# Autodesk Inventor assembly: FE-00002-11
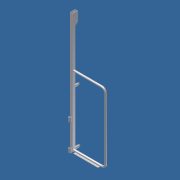
[picture p0: Inventor's stored thumbnail of the model, 180x180]
Saved by Autodesk Inventor 2012 (Build 160160000, 160)
## iProperties
Created: 2008-05-15
Part Number: FE-00002-11
Document SubType Name: Assembly
Designer: narosenberg
Author: narosenberg
## Documents named in this file (8)
- C:\Data Folder\FRC 2012 Field\Components\FE-00002-11.iam
- C:\Data Folder\FRC 2012 Field\Components\FE-00002-01.ipt
- C:\Data Folder\FRC 2012 Field\Components\FE-00002-02.ipt
- C:\Data Folder\FRC 2012 Field\Components\FE-00002-03.ipt
- C:\Data Folder\FRC 2012 Field\Components\FE-00002-05.ipt
- C:\Data Folder\FRC 2012 Field\Components\FE-00002-06.ipt
- C:\Data Folder\FRC 2012 Field\Components\FE-00002-07.ipt
- C:\Data Folder\FRC 2012 Field\Components\FE-00002-09.ipt
## Components (8 placed, 7 different names)
1. FE-00002-06:1 — Mate:1, Tangent:1, Flush:1, Mate:4
2. FE-00002-07:1 — Mate:3, Tangent:1, Flush:1, Flush:2
3. FE-00002-05:1 — Mate:4, Flush:2, Flush:3, Insert:1, Insert:2, Mate:6, Mate:7, Mate:8, Mate:9, Tangent:2, Flush:4
4. FE-00002-01:1 — Insert:1
5. FE-00002-02:1 — Insert:2
6. FE-00002-03:1 — Mate:6, Mate:7
7. FE-00002-09:2 — Mate:12, Tangent:2, Flush:4, Insert:3
8. FE-00002-09:1 — Mate:13, Insert:3
## Relationships (24: Mate 14, Flush 4, Insert 3, Tangent 2, Angle 1)
- Mate:1: FE-00002-06:1
- Mate:2
- Angle:1 (90 deg)
- Mate:3: FE-00002-07:1
- Tangent:1: FE-00002-06:1 ↔ FE-00002-07:1
- Flush:1 (25.4 mm): FE-00002-06:1 ↔ FE-00002-07:1
- Mate:4: FE-00002-06:1 ↔ FE-00002-05:1
- Flush:2: FE-00002-07:1 ↔ FE-00002-05:1
- Flush:3 (-22.225 mm): FE-00002-05:1
- Mate:5
- Insert:1: FE-00002-05:1 ↔ FE-00002-01:1
- Insert:2: FE-00002-05:1 ↔ FE-00002-02:1
- Mate:6: FE-00002-05:1 ↔ FE-00002-03:1
- Mate:7: FE-00002-05:1 ↔ FE-00002-03:1
- Mate:8: FE-00002-05:1
- Mate:9: FE-00002-05:1
- Mate:10
- Mate:11
- Mate:12: FE-00002-09:2
- Mate:13: FE-00002-09:1
- Mate:14
- Tangent:2: FE-00002-05:1 ↔ FE-00002-09:2
- Flush:4: FE-00002-05:1 ↔ FE-00002-09:2
- Insert:3 (441.325 mm): FE-00002-09:2 ↔ FE-00002-09:1
